# Autodesk Inventor assembly: Track Design 9-24-19
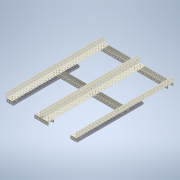
[picture p0: Inventor's stored thumbnail of the model, 180x180]
Saved by Autodesk Inventor 2020 (Build 240168000, 168)
## iProperties
Created: 2019-07-25
Part Number: Track Design 9-24-19
Document SubType Name: Assembly
Designer: Corey
Author: Corey
## Documents named in this file (7)
- C:\Users\Corey\Documents\Tower-Takeover-CAD\Parts\Dual Track.iam
- C:\Users\Corey\Documents\Tower-Takeover-CAD\Parts\Structure\90 Degree Brackets\Aluminum\Aluminum Angle 2x2x35.ipt
- C:\Users\Corey\Documents\Tower-Takeover-CAD\Parts\Cube.iam
- C:\Users\Corey\Documents\Tower-Takeover-CAD\Parts\Structure\C-Channels\Aluminum\2-Wide\Aluminum C-Channel 1x2x1x25.ipt
- C:\Users\Corey\Documents\Tower-Takeover-CAD\Parts\Structure\C-Channels\Aluminum\2-Wide\Aluminum C-Channel 1x2x1x5.ipt
- C:\Users\Corey\Documents\Tower-Takeover-CAD\Parts\Structure\C-Channels\Aluminum\2-Wide\Aluminum C-Channel 1x2x1x2.ipt
- C:\Users\Corey\Documents\Tower-Takeover-CAD\Parts\Motion\12'' Long Linear Slide Track.ipt
## Components (13 placed, 6 different names)
1. Aluminum Angle 2x2x35:1 — Flush:4, Flush:5, Flush:6, Mate:2, Flush:13, Flush:14, Mate:4, Flush:17, Flush:18, Flush:23, Flush:24
2. Aluminum Angle 2x2x35:2 — Flush:1, Flush:2, Flush:3, Flush:9, Flush:10
3. Aluminum Angle 2x2x35:3 — Flush:1, Flush:2, Flush:4, Mate:1, Flush:11, Flush:12, Mate:3, Flush:15, Flush:16
4. Aluminum Angle 2x2x35:4 — Flush:3, Flush:7, Flush:8, Mate:5, Flush:19, Flush:20, Flush:21, Flush:22
5. Cube:1 [sub-assembly]
6. Cube:2 [sub-assembly]
7. Aluminum C-Channel 1x2x1x25:1 — Mate:2, Flush:13, Flush:14
8. Aluminum C-Channel 1x2x1x25:3 — Mate:1, Flush:5, Flush:6, Flush:7, Flush:8, Flush:9, Flush:10, Flush:11, Flush:12
9. Aluminum C-Channel 1x2x1x5:1 — Mate:3, Flush:15, Flush:16
10. Aluminum C-Channel 1x2x1x2:1 — Mate:4, Flush:17, Flush:18, Mate:7
11. Aluminum C-Channel 1x2x1x2:2 — Mate:5, Flush:19, Flush:20, Mate:6
12. 12'' Long Linear Slide Track:1 — Mate:7, Flush:23, Flush:24
13. 12'' Long Linear Slide Track:2 — Mate:6, Flush:21, Flush:22
## Relationships (31: Flush 24, Mate 7)
- Flush:1: Aluminum Angle 2x2x35:2 ↔ Aluminum Angle 2x2x35:3
- Flush:2: Aluminum Angle 2x2x35:2 ↔ Aluminum Angle 2x2x35:3
- Flush:3: Aluminum Angle 2x2x35:2 ↔ Aluminum Angle 2x2x35:4
- Flush:4: Aluminum Angle 2x2x35:1 ↔ Aluminum Angle 2x2x35:3
- Mate:1: Aluminum Angle 2x2x35:3 ↔ Aluminum C-Channel 1x2x1x25:3
- Flush:5: Aluminum Angle 2x2x35:1 ↔ Aluminum C-Channel 1x2x1x25:3
- Flush:6: Aluminum Angle 2x2x35:1 ↔ Aluminum C-Channel 1x2x1x25:3
- Flush:7: Aluminum Angle 2x2x35:4 ↔ Aluminum C-Channel 1x2x1x25:3
- Flush:8: Aluminum Angle 2x2x35:4 ↔ Aluminum C-Channel 1x2x1x25:3
- Flush:9: Aluminum Angle 2x2x35:2 ↔ Aluminum C-Channel 1x2x1x25:3
- Flush:10: Aluminum Angle 2x2x35:2 ↔ Aluminum C-Channel 1x2x1x25:3
- Flush:11: Aluminum Angle 2x2x35:3 ↔ Aluminum C-Channel 1x2x1x25:3
- Flush:12: Aluminum Angle 2x2x35:3 ↔ Aluminum C-Channel 1x2x1x25:3
- Mate:2: Aluminum Angle 2x2x35:1 ↔ Aluminum C-Channel 1x2x1x25:1
- Flush:13: Aluminum Angle 2x2x35:1 ↔ Aluminum C-Channel 1x2x1x25:1
- Flush:14: Aluminum Angle 2x2x35:1 ↔ Aluminum C-Channel 1x2x1x25:1
- Mate:3: Aluminum Angle 2x2x35:3 ↔ Aluminum C-Channel 1x2x1x5:1
- Flush:15: Aluminum Angle 2x2x35:3 ↔ Aluminum C-Channel 1x2x1x5:1
- Flush:16: Aluminum Angle 2x2x35:3 ↔ Aluminum C-Channel 1x2x1x5:1
- Mate:4: Aluminum Angle 2x2x35:1 ↔ Aluminum C-Channel 1x2x1x2:1
- Mate:5: Aluminum Angle 2x2x35:4 ↔ Aluminum C-Channel 1x2x1x2:2
- Flush:17: Aluminum Angle 2x2x35:1 ↔ Aluminum C-Channel 1x2x1x2:1
- Flush:18: Aluminum Angle 2x2x35:1 ↔ Aluminum C-Channel 1x2x1x2:1
- Flush:19: Aluminum Angle 2x2x35:4 ↔ Aluminum C-Channel 1x2x1x2:2
- Flush:20: Aluminum Angle 2x2x35:4 ↔ Aluminum C-Channel 1x2x1x2:2
- Mate:6: Aluminum C-Channel 1x2x1x2:2 ↔ 12'' Long Linear Slide Track:2
- Mate:7: Aluminum C-Channel 1x2x1x2:1 ↔ 12'' Long Linear Slide Track:1
- Flush:21: Aluminum Angle 2x2x35:4 ↔ 12'' Long Linear Slide Track:2
- Flush:22: Aluminum Angle 2x2x35:4 ↔ 12'' Long Linear Slide Track:2
- Flush:23: Aluminum Angle 2x2x35:1 ↔ 12'' Long Linear Slide Track:1
- Flush:24: Aluminum Angle 2x2x35:1 ↔ 12'' Long Linear Slide Track:1
